# Autodesk Inventor assembly: ASY PNS 1750 filter-distribution-system 1200
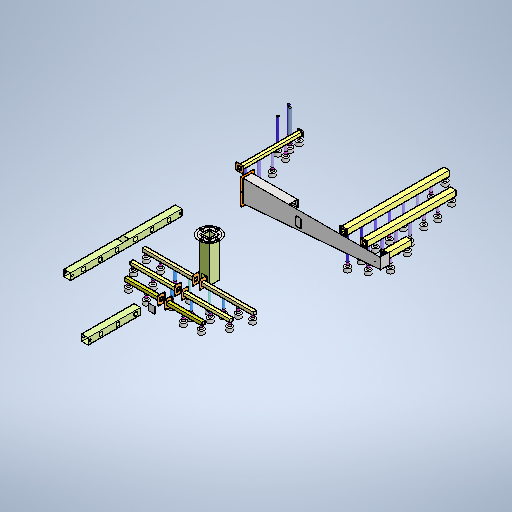
[picture p0: Inventor's stored thumbnail of the model, 512x512]
Saved by Autodesk Inventor 2025 (Build 290162010, 162A)
## iProperties
Created: 2025-06-24
Part Number: ASY PNS 1750 filter-distribution-system 1200
Document SubType Name: Assembly
Designer: user
Author: user
## Documents named in this file (14)
- C:\Users\admin\Yandex.Disk\home pc\Inventor\ANP--Antipayuta\ASY PNS 1750 filter-distribution-system 1200.iam
- C:\Users\admin\Yandex.Disk\home pc\Inventor\ANP--Antipayuta\Workspaces\Workspace\filter-distribution-system\PNS 1759 DIM filter-distribution-system 1200.ipt
- C:\Users\admin\Yandex.Disk\home pc\Inventor\ANP--Antipayuta\Workspaces\Workspace\filter-distribution-system\PNS 754 FDS 1200 FLANGE.ipt
- C:\Users\admin\Yandex.Disk\home pc\Inventor\ANP--Antipayuta\Workspaces\Workspace\filter-distribution-system\PNS 752 FDS 1200 FLANGE 2.ipt
- C:\Users\admin\Yandex.Disk\home pc\Inventor\ANP--Antipayuta\PNS 753 FDS 1200 FLANGE 3.ipt
- C:\Users\admin\Yandex.Disk\home pc\Inventor\ANP--Antipayuta\Workspaces\Workspace\filter-distribution-system\ASY PNS FDS way1.iam
- C:\Users\admin\Yandex.Disk\home pc\Inventor\ANP--Antipayuta\Workspaces\Workspace\filter-distribution-system\ASY PNS 1752 FDS way 2.iam
- C:\Users\admin\Yandex.Disk\home pc\Inventor\ANP--Antipayuta\Workspaces\Workspace\filter-distribution-system\ASY PNS FDS way3.iam
- C:\Users\admin\Yandex.Disk\home pc\Inventor\ANP--Antipayuta\PNS 767 FDS 1200 CUP 2.ipt
- C:\Users\admin\Yandex.Disk\home pc\Inventor\ANP--Antipayuta\PNS 765 FDS 1200 CUP 1.ipt
- C:\Users\admin\Yandex.Disk\home pc\Inventor\ANP--Antipayuta\PNS 1757 FDS 1200x50 FLANGE.ipt
- C:\Users\admin\Yandex.Disk\home pc\Inventor\ANP--Antipayuta\PNS 1761 FDS 1200x50 central way.ipt
- C:\Users\admin\Yandex.Disk\home pc\Inventor\ANP--Antipayuta\PNS 1762 FDS 1200x50 column.ipt
- C:\Users\admin\Yandex.Disk\home pc\Inventor\ANP--Antipayuta\FDS 1400\ASY ANP 1490 FDS one way.iam
## Components (17 placed, 13 different names)
1. PNS 751 DIM filter-distribution-system 1200.ipt:1 — Mate:4, Mate:5
2. PNS 754 FDS 1200 FLANGE.ipt:1 — Mate:1, Flush:1, Flush:2
3. PNS 752 FDS 1200 FLANGE 2.ipt:1 — Rigid:1, Flush:1, Mate:6, Flush:3, Flush:4
4. PNS 752 FDS 1200 FLANGE 2.ipt:2 — Rigid:1, Mate:1, Flush:2
5. PNS 753 FDS 1200 FLANGE 3.ipt:2
6. ASY PNS FDS way1.iam:3 [sub-assembly]
7. ASY PNS FDS way1.iam:4 [sub-assembly]
8. ASY PNS FDS way 2.iam:3 [sub-assembly]
9. ASY PNS FDS way 2.iam:4 [sub-assembly]
10. ASY PNS FDS way3.iam:3 [sub-assembly]
11. ASY PNS FDS way3.iam:4 [sub-assembly]
12. PNS 767 FDS 1200 CUP 2.ipt:1
13. PNS 765 FDS 1200 CUP 1.ipt:1 — Mate:6, Flush:3, Flush:4
14. PNS 1757 FDS 1200x50 FLANGE:1 — Rigid:35, Flush:5, Mate:7, Flush:6
15. PNS 1761 FDS 1200x50 central way:1
16. PNS 1762 FDS 1200x50 column:1 — Rigid:35
17. ASY ANP 1490 FDS one way:1 [sub-assembly]
## Relationships (13: Flush 6, Mate 5, WeldJoint 2)
- Rigid:1 [WeldJoint]: PNS 752 FDS 1200 FLANGE 2.ipt:1 ↔ PNS 752 FDS 1200 FLANGE 2.ipt:2
- Mate:1: PNS 754 FDS 1200 FLANGE.ipt:1 ↔ PNS 752 FDS 1200 FLANGE 2.ipt:2
- Flush:1: PNS 754 FDS 1200 FLANGE.ipt:1 ↔ PNS 752 FDS 1200 FLANGE 2.ipt:1
- Flush:2: PNS 754 FDS 1200 FLANGE.ipt:1 ↔ PNS 752 FDS 1200 FLANGE 2.ipt:2
- Mate:4: PNS 751 DIM filter-distribution-system 1200.ipt:1
- Mate:5: PNS 751 DIM filter-distribution-system 1200.ipt:1
- Mate:6: PNS 752 FDS 1200 FLANGE 2.ipt:1 ↔ PNS 765 FDS 1200 CUP 1.ipt:1
- Flush:3: PNS 752 FDS 1200 FLANGE 2.ipt:1 ↔ PNS 765 FDS 1200 CUP 1.ipt:1
- Flush:4: PNS 752 FDS 1200 FLANGE 2.ipt:1 ↔ PNS 765 FDS 1200 CUP 1.ipt:1
- Rigid:35 [WeldJoint]: PNS 1757 FDS 1200x50 FLANGE:1 ↔ PNS 1762 FDS 1200x50 column:1
- Flush:5: PNS 1757 FDS 1200x50 FLANGE:1
- Mate:7: PNS 1757 FDS 1200x50 FLANGE:1
- Flush:6: PNS 1757 FDS 1200x50 FLANGE:1
